# Autodesk Inventor assembly: KALM_05_CL_1
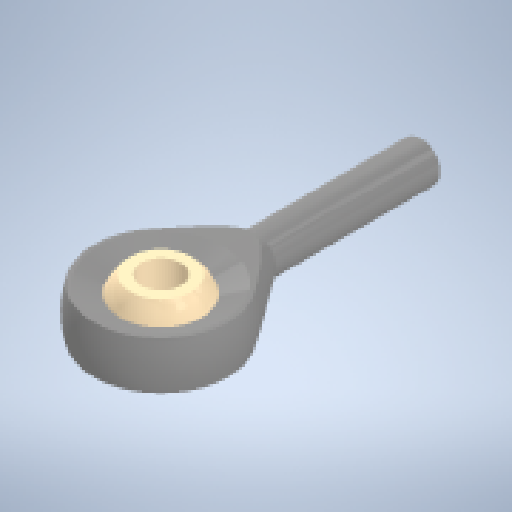
[picture p0: Inventor's stored thumbnail of the model, 512x512]
Saved by Autodesk Inventor 2025.4 (Build 294407000, 407)
## iProperties
Company: CADClick - www.CADClick.com
Created: 2026-05-12
Part Number: KALM_05_CL_1
Description: STEP AP214
Document SubType Name: Assembly
Designer: louis
Authority: unknown authorization
Preprocessor: Spatial InterOp 3D
Title: cctmp_BE5C459D-53DB-43ED-8152-0BDBA59D5F99_2026_05_12_10_23_57_0867_133736..stp
Author: igus GmbH
## Documents named in this file (4)
- C:\Users\louis\OneDrive\Desktop\R_Trident\02_CAD\01_Standard_Parts\KALM_05_CL_1\KALM_05_CL_1\KALM_05_CL_1.iam
- C:\Users\louis\OneDrive\Desktop\R_Trident\02_CAD\01_Standard_Parts\KALM_05_CL_1\KALM_05_CL_1\2026_05_12_10_23_57_0836.ipt
- C:\Users\louis\OneDrive\Desktop\R_Trident\02_CAD\01_Standard_Parts\KALM_05_CL_1\KALM_05_CL_1\2026_05_12_10_23_57_0851.ipt
- C:\Users\louis\OneDrive\Desktop\R_Trident\02_CAD\01_Standard_Parts\KALM_05_CL_1\KALM_05_CL_1\2026_05_12_10_23_57_0867.ipt
## Components (3 placed, 3 different names)
1. 2026_05_12_10_23_57_0836
2. 2026_05_12_10_23_57_0851 — Mate:1, Angle:1, Mate:2, Ball:1
3. 2026_05_12_10_23_57_0867 — Mate:1, Angle:1, Mate:2, Ball:1
## Relationships (4: Mate 2, Angle 1, BallJoint 1)
- Mate:1: 2026_05_12_10_23_57_0851 ↔ 2026_05_12_10_23_57_0867
- Angle:1 (35 deg): 2026_05_12_10_23_57_0851 ↔ 2026_05_12_10_23_57_0867
- Mate:2: 2026_05_12_10_23_57_0851 ↔ 2026_05_12_10_23_57_0867
- Ball:1: 2026_05_12_10_23_57_0851 ↔ 2026_05_12_10_23_57_0867
